# Autodesk Inventor assembly: FYP-Assembly
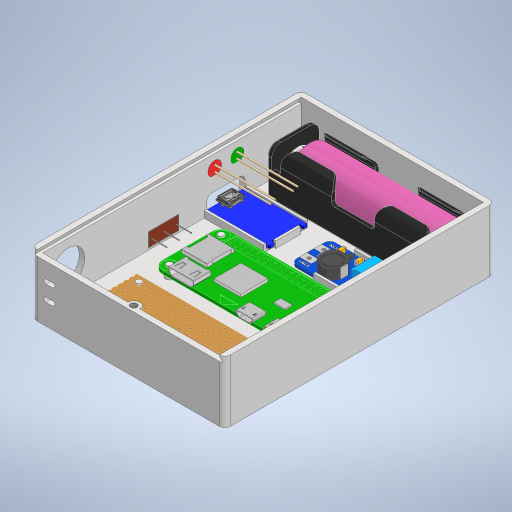
[picture p0: Inventor's stored thumbnail of the model, 512x512]
Saved by Autodesk Inventor 2023 (Build 270158000, 158)
## iProperties
Created: 2024-02-14
Part Number: FYP-Assembly
Document SubType Name: Assembly
Designer: ongyu
Author: ongyu
## Documents named in this file (13)
- C:\Users\ongyu\OneDrive\Documents\Inventor\FYP\Electronic-Enclosure\Compartment-Assembly-old.iam
- C:\Users\ongyu\OneDrive\Documents\Inventor\FYP\Electronic-Enclosure\01-Electronic-Compartment.ipt
- C:\Users\ongyu\OneDrive\Documents\Inventor\FYP\Electronic-Enclosure\04-RaspberryPiZeroW.ipt
- C:\Users\ongyu\OneDrive\Documents\Inventor\FYP\Electronic-Enclosure\02-18650-Battery-Holder.ipt
- C:\Users\ongyu\OneDrive\Documents\Inventor\FYP\Electronic-Enclosure\05-TP_4056.ipt
- C:\Users\ongyu\OneDrive\Documents\Inventor\FYP\Electronic-Enclosure\03-MT3608-Module.ipt
- C:\Users\ongyu\OneDrive\Documents\Inventor\FYP\Electronic-Enclosure\07-Green-LED-5mm.ipt
- C:\Users\ongyu\OneDrive\Documents\Inventor\FYP\Electronic-Enclosure\06-Red-LED-5mm.ipt
- C:\Users\ongyu\OneDrive\Documents\Inventor\FYP\Electronic-Enclosure\09-18650-Battery.ipt
- C:\Users\ongyu\OneDrive\Documents\Inventor\FYP\Electronic-Enclosure\11-Small-Switch.ipt
- C:\Users\ongyu\OneDrive\Documents\Inventor\FYP\Electronic-Enclosure\10-Stripboard.ipt
- C:\Users\ongyu\OneDrive\Documents\Inventor\FYP\12-Electronic-Compartment-Cover.ipt
- C:\Users\ongyu\OneDrive\Documents\Inventor\FYP\12-5-Electronic-Compartment-Cover-Holes.ipt
## Components (12 placed, 12 different names)
1. 01-Electronic-Compartment:1 — Mate:1, Flush:3, Flush:5, Flush:6, Mate:6, Insert:1, Insert:2, Mate:7, Mate:11, Mate:12, Flush:7, Mate:13, Mate:14, Mate:15, Insert:6, Insert:7, Mate:16, Mate:17, Mate:18, Mate:19, Mate:21, Insert:8, Insert:9
2. 04-RaspberryPiZeroW:1 — Insert:1, Insert:2
3. 02-18650-Battery-Holder:1 — Mate:1, Mate:6, Insert:5, Mate:21
4. 05-TP_4056:1 — Mate:7, Mate:18
5. 03-MT3608-Module:1 — Mate:15
6. 07-Green-LED-5mm:1 — Insert:7, Mate:17
7. 06-Red-LED-5mm:1 — Insert:6, Mate:16
8. 09-18650-Battery:1 — Insert:5
9. 11-Small-Switch:1 — Mate:11, Mate:12, Flush:7
10. 10-Stripboard:1 — Insert:8, Insert:9
11. 12-Electronic-Compartment-Cover:1 — Mate:13, Mate:14
12. 12-5-Electronic-Compartment-Cover-Holes:1 — Mate:19
## Relationships (24: Mate 13, Insert 7, Flush 4)
- Mate:1: 01-Electronic-Compartment:1 ↔ 02-18650-Battery-Holder:1
- Flush:3: 01-Electronic-Compartment:1
- Flush:5: 01-Electronic-Compartment:1
- Flush:6: 01-Electronic-Compartment:1
- Mate:6: 01-Electronic-Compartment:1 ↔ 02-18650-Battery-Holder:1
- Insert:1: 01-Electronic-Compartment:1 ↔ 04-RaspberryPiZeroW:1
- Insert:2: 01-Electronic-Compartment:1 ↔ 04-RaspberryPiZeroW:1
- Mate:7: 01-Electronic-Compartment:1 ↔ 05-TP_4056:1
- Insert:5: 02-18650-Battery-Holder:1 ↔ 09-18650-Battery:1
- Mate:11 (0.25 mm): 01-Electronic-Compartment:1 ↔ 11-Small-Switch:1
- Mate:12 (0.25 mm): 01-Electronic-Compartment:1 ↔ 11-Small-Switch:1
- Flush:7: 01-Electronic-Compartment:1 ↔ 11-Small-Switch:1
- Mate:13: 01-Electronic-Compartment:1 ↔ 12-Electronic-Compartment-Cover:1
- Mate:14: 01-Electronic-Compartment:1 ↔ 12-Electronic-Compartment-Cover:1
- Mate:15: 01-Electronic-Compartment:1 ↔ 03-MT3608-Module:1
- Insert:6: 01-Electronic-Compartment:1 ↔ 06-Red-LED-5mm:1
- Insert:7: 01-Electronic-Compartment:1 ↔ 07-Green-LED-5mm:1
- Mate:16: 01-Electronic-Compartment:1 ↔ 06-Red-LED-5mm:1
- Mate:17: 01-Electronic-Compartment:1 ↔ 07-Green-LED-5mm:1
- Mate:18: 01-Electronic-Compartment:1 ↔ 05-TP_4056:1
- Mate:19: 01-Electronic-Compartment:1 ↔ 12-5-Electronic-Compartment-Cover-Holes:1
- Mate:21: 01-Electronic-Compartment:1 ↔ 02-18650-Battery-Holder:1
- Insert:8: 01-Electronic-Compartment:1 ↔ 10-Stripboard:1
- Insert:9: 01-Electronic-Compartment:1 ↔ 10-Stripboard:1
